# Autodesk Inventor assembly: RB12
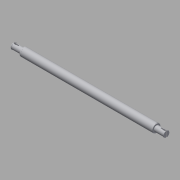
[picture p0: Inventor's stored thumbnail of the model, 180x180]
Saved by Autodesk Inventor 2019.3 (Build 233278000, 278)
## iProperties
Created: 2019-02-05
Part Number: RB12
Document SubType Name: Assembly
Designer: Varga Daniel
Author: Varga Daniel
## Documents named in this file (6)
- C:\!_Dani\!_cloud\OneDrive\!_munka\Revolution\RevvyDemoKit\Structural parts\Beams\Round Beams\RB1+\RB12.iam
- C:\!_Dani\!_cloud\OneDrive\!_munka\Revolution\RevvyDemoKit\Structural parts\Beams\Round Beams\Round_beam_body.ipt
- C:\!_Dani\!_cloud\OneDrive\!_munka\Revolution\RevvyDemoKit\Structural parts\Connetor Pins\Connector_pin_collar.ipt
- C:\!_Dani\!_cloud\OneDrive\!_munka\Revolution\RevvyDemoKit\Structural parts\Connetor Pins\Connector_pin_stick.ipt
- C:\!_Dani\!_cloud\OneDrive\!_munka\Revolution\RevvyDemoKit\Structural parts\Beams\Round Beams\RB1+.iam
- C:\!_Dani\!_cloud\OneDrive\!_munka\Revolution\RevvyDemoKit\Structural parts\Beams\Round Beams\Round_beam_body\Round_beam_body-12.ipt
## Components (5 placed, 3 different names)
1. Round_beam_body-12:1 — Mate:5, Mate:6, Mate:7, Mate:8
2. Connector_pin_collar:1 — Mate:3, Mate:4, Mate:5, Mate:6
3. Connector_pin_stick:1 — Mate:3, Mate:4, Angle:1
4. Connector_pin_collar:2 — Mate:1, Mate:2, Mate:7, Mate:8
5. Connector_pin_stick:2 — Mate:1, Mate:2, Angle:1, Angle:2
## Relationships (10: Mate 8, Angle 2)
- Mate:1: Connector_pin_collar:2 ↔ Connector_pin_stick:2
- Mate:2: Connector_pin_collar:2 ↔ Connector_pin_stick:2
- Mate:3: Connector_pin_collar:1 ↔ Connector_pin_stick:1
- Mate:4: Connector_pin_collar:1 ↔ Connector_pin_stick:1
- Mate:5: Round_beam_body-12:1 ↔ Connector_pin_collar:1
- Mate:6: Round_beam_body-12:1 ↔ Connector_pin_collar:1
- Mate:7: Round_beam_body-12:1 ↔ Connector_pin_collar:2
- Mate:8: Round_beam_body-12:1 ↔ Connector_pin_collar:2
- Angle:1 (0 deg): Connector_pin_stick:1 ↔ Connector_pin_stick:2
- Angle:2 (0 deg): Connector_pin_stick:2
